# Autodesk Inventor assembly: Aircraft Preliminary Design and W+B
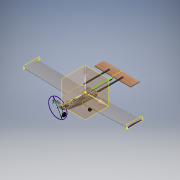
[picture p0: Inventor's stored thumbnail of the model, 180x180]
Saved by Autodesk Inventor 2018 (Build 220112000, 112)
## iProperties
Created: 2018-07-21
Part Number: Aircraft Preliminary Design and W+B
Document SubType Name: Assembly
Designer: Michael Gunderman
Mass: 3069.82 g
Surface Area: 15344.9 cm^2
Volume: 13743.9 cm^3
Density: 0.223358 g/cm^3
Author: Michael Gunderman
## Documents named in this file (12)
- C:\Users\Michael Gunderman\Downloads\Aircraft Preliminary Design and W+B.iam
- C:\Users\Michael Gunderman\Documents\Special Projects\Echo 1\CAD work\Systems\Electrical\Motor Turnigy G60 500kv.ipt
- C:\Users\Michael Gunderman\Downloads\Generic Wing 1.ipt
- C:\Users\Michael Gunderman\Downloads\Generic Tail 1.ipt
- C:\Users\Michael Gunderman\Documents\Special Projects\Echo 1\CAD work\Structures\500mm tube.ipt
- C:\Users\Michael Gunderman\Documents\Special Projects\Echo 1\CAD work\Structures\500mm tube_MIR.ipt
- C:\Users\Michael Gunderman\Documents\Special Projects\Echo 1\CAD work\Systems\Electrical\Flight Battery 5000 mah 5S.ipt
- C:\Users\Michael Gunderman\Downloads\Generic Wing 1_MIR2.ipt
- C:\Users\Michael Gunderman\Documents\Special Projects\Echo 1\CAD work\Preliminary Shapes\Main Landing Gear.ipt
- C:\Users\Michael Gunderman\Documents\Special Projects\Echo 1\CAD work\Systems\Landing Gear\Nose Gear Assembly.iam
- C:\Users\Michael Gunderman\Documents\Special Projects\Echo 1\CAD work\Systems\Payload\Bravo 1 Mockup.ipt
- C:\Users\Michael Gunderman\Documents\Special Projects\Echo 1\CAD work\Preliminary Shapes\Generic Fuselage.ipt
## Components (12 placed, 11 different names)
1. Motor Turnigy G60 500kv:1 — Mate:4
2. Generic Wing 1:1 — Mate:1
3. Generic Tail 1:1 — Mate:2
4. 500mm tube:1
5. 500mm tube_MIR:1
6. Flight Battery 5000 mah 5S:1
7. Generic Wing 1_MIR2:1 — Mate:3
8. Main Landing Gear:1
9. Main Landing Gear:2
10. Nose Gear Assembly:1 [sub-assembly]
11. Bravo 1 Mockup:1
12. Generic Fuselage:1
## Relationships (5: Mate 4, Flush 1)
- Flush:1 (143 mm)
- Mate:1: Generic Wing 1:1
- Mate:2: Generic Tail 1:1
- Mate:3: Generic Wing 1_MIR2:1
- Mate:4: Motor Turnigy G60 500kv:1
